# Autodesk Inventor assembly: Zespół
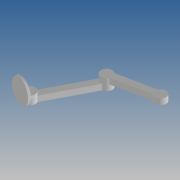
[picture p0: Inventor's stored thumbnail of the model, 180x180]
Saved by Autodesk Inventor 2022.3 (Build 263350000, 350)
## iProperties
Created: 2023-06-25
Part Number: Zespół
Document SubType Name: Assembly
Designer: Chyba Ja
Author: Chyba Ja
## Documents named in this file (4)
- C:\Users\Chyba Ja\Documents\Inventor\WALL-E\Zespół.iam
- C:\Users\Chyba Ja\Documents\Inventor\WALL-E\1stopien.ipt
- C:\Users\Chyba Ja\Documents\Inventor\WALL-E\2stopien.ipt
- C:\Users\Chyba Ja\Documents\Inventor\WALL-E\podstawa.ipt
## Components (3 placed, 3 different names)
1. 1stopien:1 — Zestawiające:1, Zestawiające:2, Zestawiające:3, Zestawiające:4
2. 2stopien:1 — Zestawiające:1, Zestawiające:2
3. podstawa:1 — Zestawiające:3, Zestawiające:4
## Relationships (4: Mate 4)
- Zestawiające:1 [Mate]: 1stopien:1 ↔ 2stopien:1
- Zestawiające:2 [Mate]: 1stopien:1 ↔ 2stopien:1
- Zestawiające:3 [Mate]: 1stopien:1 ↔ podstawa:1
- Zestawiające:4 [Mate]: 1stopien:1 ↔ podstawa:1
